# Autodesk Inventor assembly: 3A.01.13.JS.Rib 13
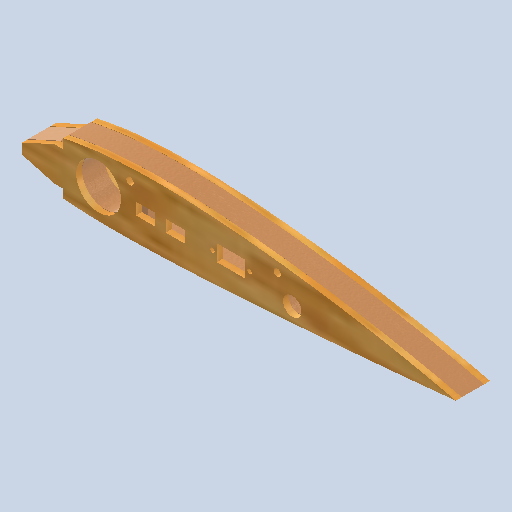
[picture p0: Inventor's stored thumbnail of the model, 512x512]
Saved by Autodesk Inventor 2025.1 (Build 291241000, 241)
## iProperties
Created: 2025-01-14
Part Number: 3A.01.13.JS.Rib 13
Document SubType Name: Assembly
Designer: johan
Author: johan
## Documents named in this file (4)
- C:\Users\johan\OneDrive - University of Bristol\CAD docs\2) Wing\2) Ribs\assemblies\3A.01.13.JS.Rib 13.iam
- C:\Users\johan\OneDrive - University of Bristol\CAD docs\2) Wing\2) Ribs\parts\Full length unmodified\3P.03.13.01.JS.rib 13 ply.ipt
- C:\Users\johan\OneDrive - University of Bristol\CAD docs\2) Wing\2) Ribs\parts\Full length unmodified\3P.03.13.02.JS.rib 13 foam.ipt
- C:\Users\johan\OneDrive - University of Bristol\CAD docs\2) Wing\2) Ribs\parts\Full length unmodified\3P.03.13.03.JS.rib 13 ply avionics cuttout.ipt
## Components (3 placed, 3 different names)
1. 3P.03.13.02.JS.rib 13 foam:1 — Rigid:2, Rigid:3
2. 3P.03.13.01.JS.rib 13 ply:2 — Rigid:2
3. 3P.03.13.03.JS.rib 13 ply avionics cuttout:1 — Rigid:3
## Relationships (2: WeldJoint 2)
- Rigid:2 [WeldJoint]: 3P.03.13.02.JS.rib 13 foam:1 ↔ 3P.03.13.01.JS.rib 13 ply:2
- Rigid:3 [WeldJoint]: 3P.03.13.02.JS.rib 13 foam:1 ↔ 3P.03.13.03.JS.rib 13 ply avionics cuttout:1
